# Autodesk Inventor assembly: base
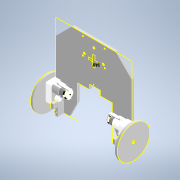
[picture p0: Inventor's stored thumbnail of the model, 180x180]
Saved by Autodesk Inventor 2020.1 (Build 241239000, 239)
## iProperties
Created: 2019-10-30
Part Number: base
Document SubType Name: Assembly
Designer: amirs
Author: amirs
## Documents named in this file (7)
- C:\Users\amirs\Downloads\base.iam
- C:\Users\amirs\Downloads\BoardProj.ipt
- C:\Users\amirs\Downloads\WheelProj.ipt
- C:\Users\amirs\Downloads\MotorHolder 2.ipt
- C:\Users\amirs\Downloads\Solarbotics-GM2_Assem.iam
- C:\Users\amirs\Downloads\PegAssembly (1).iam
- C:\Users\amirs\Downloads\WheelCap.ipt
## Components (10 placed, 6 different names)
1. BoardProj:1 — Mate:1, Mate:2, Mate:3, Mate:6, Mate:7, Mate:8, Mate:15, Mate:21, Mate:22
2. WheelProj:1 — Mate:23, Mate:31
3. WheelProj:2 — Mate:12, Mate:28
4. MotorHolder 2:1 — Mate:1, Mate:2, Mate:3, Mate:24, Mate:25
5. MotorHolder 2:2 — Mate:6, Mate:7, Mate:8, Mate:9, Mate:10, Mate:11
6. Solarbotics-GM2_Assem:1 [sub-assembly] — Mate:9, Mate:10, Mate:11, Mate:12, Mate:26, Mate:27
7. PegAssembly (1):1 [sub-assembly] — Mate:15, Mate:21, Mate:22
8. Solarbotics-GM2_Assem:2 [sub-assembly] — Mate:23, Mate:24, Mate:25, Mate:29, Mate:30
9. WheelCap:1 — Mate:26, Mate:27, Mate:28
10. WheelCap:2 — Mate:29, Mate:30, Mate:31
## Relationships (22: Mate 22)
- Mate:1: BoardProj:1 ↔ MotorHolder 2:1
- Mate:2: BoardProj:1 ↔ MotorHolder 2:1
- Mate:3: BoardProj:1 ↔ MotorHolder 2:1
- Mate:6: BoardProj:1 ↔ MotorHolder 2:2
- Mate:7: BoardProj:1 ↔ MotorHolder 2:2
- Mate:8: BoardProj:1 ↔ MotorHolder 2:2
- Mate:9: MotorHolder 2:2 ↔ Solarbotics-GM2_Assem:1
- Mate:10: MotorHolder 2:2 ↔ Solarbotics-GM2_Assem:1
- Mate:11: MotorHolder 2:2 ↔ Solarbotics-GM2_Assem:1
- Mate:12: WheelProj:2 ↔ Solarbotics-GM2_Assem:1
- Mate:15: BoardProj:1 ↔ PegAssembly (1):1
- Mate:21: BoardProj:1 ↔ PegAssembly (1):1
- Mate:22: BoardProj:1 ↔ PegAssembly (1):1
- Mate:23: WheelProj:1 ↔ Solarbotics-GM2_Assem:2
- Mate:24: MotorHolder 2:1 ↔ Solarbotics-GM2_Assem:2
- Mate:25: MotorHolder 2:1 ↔ Solarbotics-GM2_Assem:2
- Mate:26: Solarbotics-GM2_Assem:1 ↔ WheelCap:1
- Mate:27: Solarbotics-GM2_Assem:1 ↔ WheelCap:1
- Mate:28: WheelProj:2 ↔ WheelCap:1
- Mate:29: Solarbotics-GM2_Assem:2 ↔ WheelCap:2
- Mate:30: Solarbotics-GM2_Assem:2 ↔ WheelCap:2
- Mate:31: WheelProj:1 ↔ WheelCap:2
